# Autodesk Inventor assembly: EL2-400A
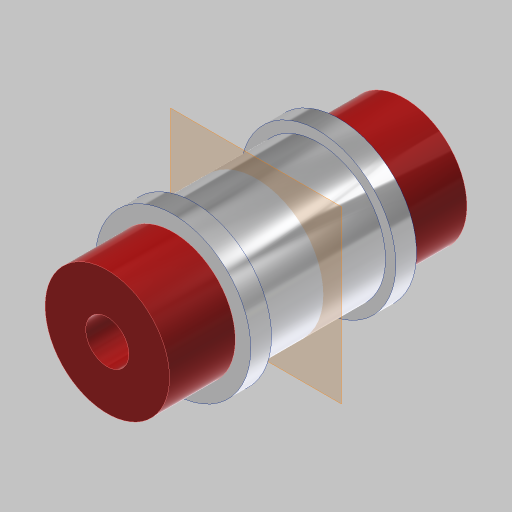
[picture p0: Inventor's stored thumbnail of the model, 512x512]
Saved by Autodesk Inventor 2023.5 (Build 275446000, 446)
## iProperties
Created: 2025-01-11
Part Number: EL2-400A
Document SubType Name: Assembly
Designer: mavericks
Author: mavericks
## Documents named in this file (4)
- C:\Users\slick\OneDrive\Desktop\2025-ReefScape---CAD\Elevator\EL2\EL2-400A.iam
- C:\Users\slick\OneDrive\Desktop\2025-ReefScape---CAD\Elevator\EL2\EL2-007.ipt
- C:\Users\slick\OneDrive\Desktop\2025-ReefScape---CAD\Elevator\EL2\EL2-401A.ipt
- C:\Users\slick\OneDrive\Desktop\2025-ReefScape---CAD\COMMON PARTS\BEARINGS\Ball Bearing 1_4x11_16x5_16 Sealed 1602DC 1602-2RS.ipt
## Components (5 placed, 3 different names)
1. EL2-007:1 — Mate:1, Mate:2, Mate:3, Mate:4, Flush:1, Flush:2
2. Ball Bearing 1_4x11_16x5_16 Sealed 1602DC 1602-2RS:1 — Mate:1, Flush:1, Mate:5
3. Ball Bearing 1_4x11_16x5_16 Sealed 1602DC 1602-2RS:2 — Mate:2, Flush:2, Mate:6
4. EL2-401A:1 — Mate:4, Mate:5
5. EL2-401A:2 — Mate:3, Mate:6
## Relationships (8: Mate 6, Flush 2)
- Mate:1: EL2-007:1 ↔ Ball Bearing 1_4x11_16x5_16 Sealed 1602DC 1602-2RS:1
- Mate:2: EL2-007:1 ↔ Ball Bearing 1_4x11_16x5_16 Sealed 1602DC 1602-2RS:2
- Mate:3: EL2-007:1 ↔ EL2-401A:2
- Mate:4: EL2-007:1 ↔ EL2-401A:1
- Flush:1: EL2-007:1 ↔ Ball Bearing 1_4x11_16x5_16 Sealed 1602DC 1602-2RS:1
- Flush:2: EL2-007:1 ↔ Ball Bearing 1_4x11_16x5_16 Sealed 1602DC 1602-2RS:2
- Mate:5: Ball Bearing 1_4x11_16x5_16 Sealed 1602DC 1602-2RS:1 ↔ EL2-401A:1
- Mate:6: Ball Bearing 1_4x11_16x5_16 Sealed 1602DC 1602-2RS:2 ↔ EL2-401A:2
